# Autodesk Inventor assembly: dynamixel_pro_assembly
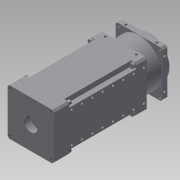
[picture p0: Inventor's stored thumbnail of the model, 180x180]
Saved by Autodesk Inventor 2017 (Build 210142000, 142)
## iProperties
Part Number: dynamixel_pro_assembly
Material: Generisch
Document SubType Name: Assembly
Designer: Max
Mass: 941.124 g
Surface Area: 510.469 cm^2
Volume: 363.722 cm^3
Density: 2.58748 g/cm^3
Author: Max
## Documents named in this file (5)
- C:\Users\Max\Desktop\SENAI\robot_arm_new\dynamixel_pro_assembly.iam
- C:\Users\Max\Desktop\SENAI\robot_arm_new\h54-200-s500-r.ipt
- C:\Users\Max\Desktop\SENAI\robot_arm_new\bearing_mount_part_2.ipt
- C:\Users\Max\Desktop\SENAI\robot_arm_new\bearing_mount_part_1.ipt
- C:\Users\Max\Documents\Inventor\Content Center Files\R2017\de-DE\DIN 912\DIN 912 - M3 x 0,5 x 16 x 14,75.ipt
## Components (7 placed, 4 different names)
1. h54-200-s500-r:1 — Passend:1, Passend:2, Passend:3, Passend:8
2. bearing_mount_part_2:1 — Passend:4, Passend:5, Passend:6, Passend:7
3. bearing_mount_part_1:1 — Passend:1, Passend:2, Passend:3, Passend:4, Passend:5, Passend:6
4. DIN 912 - ersetzt durch DIN EN ISO 4762 M3 x 16:1 — Passend:7, Passend:8
5. DIN 912 - ersetzt durch DIN EN ISO 4762 M3 x 16:2
6. DIN 912 - ersetzt durch DIN EN ISO 4762 M3 x 16:3
7. DIN 912 - ersetzt durch DIN EN ISO 4762 M3 x 16:4
## Component patterns: (4 elements, first: DIN 912 - ersetzt durch DIN EN ISO 4762 M3 x 16:1)
## Relationships (8: Mate 8)
- Passend:1 [Mate]: h54-200-s500-r:1 ↔ bearing_mount_part_1:1
- Passend:2 [Mate]: h54-200-s500-r:1 ↔ bearing_mount_part_1:1
- Passend:3 [Mate]: h54-200-s500-r:1 ↔ bearing_mount_part_1:1
- Passend:4 [Mate]: bearing_mount_part_2:1 ↔ bearing_mount_part_1:1
- Passend:5 [Mate]: bearing_mount_part_2:1 ↔ bearing_mount_part_1:1
- Passend:6 [Mate]: bearing_mount_part_2:1 ↔ bearing_mount_part_1:1
- Passend:7 [Mate]: bearing_mount_part_2:1 ↔ DIN 912 - ersetzt durch DIN EN ISO 4762 M3 x 16:1
- Passend:8 [Mate]: h54-200-s500-r:1 ↔ DIN 912 - ersetzt durch DIN EN ISO 4762 M3 x 16:1
